# Autodesk Inventor assembly: microsumno
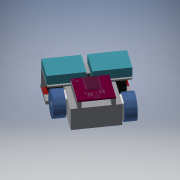
[picture p0: Inventor's stored thumbnail of the model, 180x180]
Saved by Autodesk Inventor 2016 (Build 200138000, 138)
## iProperties
Created: 2015-09-15
Part Number: microsumno
Document SubType Name: Assembly
Designer: cem
Author: cem
## Documents named in this file (8)
- C:\Users\cem\Desktop\microsumno.iam
- C:\Users\cem\Desktop\Part1.ipt
- C:\Users\cem\Desktop\mtr.ipt
- C:\Users\cem\Desktop\wheel.ipt
- C:\Users\cem\Downloads\QTR.ipt
- C:\Users\cem\Downloads\GP2Y0D340K.ipt
- C:\Users\cem\Desktop\batt.ipt
- C:\Users\cem\Desktop\kart1.ipt
## Components (13 placed, 7 different names)
1. Part1:1 — Mate:5, Mate:7, Mate:8, Mate:9, Mate:10, Mate:13, Mate:14, Mate:15, Mate:17, Mate:21, Mate:25, Mate:27, Mate:28, Mate:29, Mate:30, Mate:31, Mate:32, Mate:33, Mate:34, Mate:35, Mate:36, Mate:37, Mate:40, Mate:41, Mate:42, Mate:43, Mate:44, Mate:45, Mate:46, Mate:47
2. mtr:1 — Rotational:1, Mate:8, Mate:9, Mate:10, Mate:11, Mate:33
3. mtr:2 — Rotational:2, Mate:5, Mate:7, Mate:11
4. wheel:1 — Rotational:1
5. wheel:2 — Rotational:2
6. QTR:1 — Mate:14, Mate:15, Mate:29
7. QTR:2 — Mate:13, Mate:28, Mate:31
8. GP2Y0D340K:1 — Mate:17, Mate:21, Mate:45, Mate:46, Mate:47
9. GP2Y0D340K:2 — Mate:27, Mate:32, Mate:35
10. GP2Y0D340K:3 — Mate:25, Mate:30, Mate:36
11. batt:1 — Mate:37, Mate:43
12. batt:2 — Mate:40, Mate:44
13. kart1:1 — Mate:41, Mate:42
## Relationships (33: Mate 31, RevoluteJoint 2)
- Rotational:1 [RevoluteJoint]: mtr:1 ↔ wheel:1
- Rotational:2 [RevoluteJoint]: mtr:2 ↔ wheel:2
- Mate:5: Part1:1 ↔ mtr:2
- Mate:7: Part1:1 ↔ mtr:2
- Mate:8: Part1:1 ↔ mtr:1
- Mate:9: Part1:1 ↔ mtr:1
- Mate:10: Part1:1 ↔ mtr:1
- Mate:11: mtr:1 ↔ mtr:2
- Mate:13: Part1:1 ↔ QTR:2
- Mate:14: Part1:1 ↔ QTR:1
- Mate:15: Part1:1 ↔ QTR:1
- Mate:17: Part1:1 ↔ GP2Y0D340K:1
- Mate:21: Part1:1 ↔ GP2Y0D340K:1
- Mate:25: Part1:1 ↔ GP2Y0D340K:3
- Mate:27: Part1:1 ↔ GP2Y0D340K:2
- Mate:28: Part1:1 ↔ QTR:2
- Mate:29: Part1:1 ↔ QTR:1
- Mate:30: Part1:1 ↔ GP2Y0D340K:3
- Mate:31: Part1:1 ↔ QTR:2
- Mate:32: Part1:1 ↔ GP2Y0D340K:2
- Mate:33: Part1:1 ↔ mtr:1
- Mate:34: Part1:1
- Mate:35: Part1:1 ↔ GP2Y0D340K:2
- Mate:36: Part1:1 ↔ GP2Y0D340K:3
- Mate:37: Part1:1 ↔ batt:1
- Mate:40: Part1:1 ↔ batt:2
- Mate:41: Part1:1 ↔ kart1:1
- Mate:42: Part1:1 ↔ kart1:1
- Mate:43: Part1:1 ↔ batt:1
- Mate:44: Part1:1 ↔ batt:2
- Mate:45: Part1:1 ↔ GP2Y0D340K:1
- Mate:46: Part1:1 ↔ GP2Y0D340K:1
- Mate:47: Part1:1 ↔ GP2Y0D340K:1
